# Autodesk Inventor assembly: teljes3
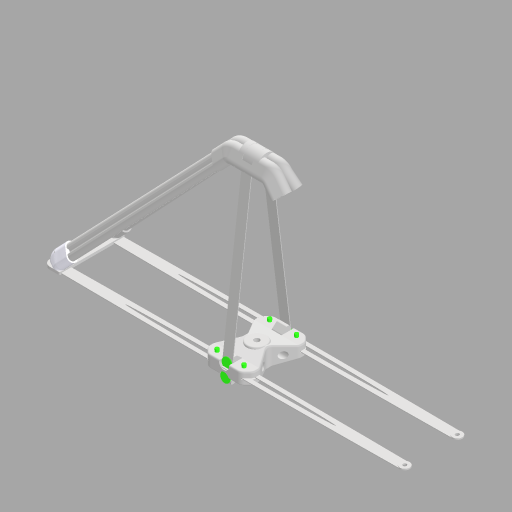
[picture p0: Inventor's stored thumbnail of the model, 512x512]
Saved by Autodesk Inventor 2023 (Build 270158000, 158)
## iProperties
Created: 2022-11-11
Part Number: teljes3
Document SubType Name: Assembly
Designer: gd1
Author: gd1
## Documents named in this file (8)
- C:\Users\gd1\3D Objects\3D nagyteherbírású híd\Híd\H-d\teljes8.iam
- C:\Users\gd1\3D Objects\3D nagyteherbírású híd\Híd\H-d\45 fok középre_talp másolata.ipt
- C:\Users\gd1\3D Objects\3D nagyteherbírású híd\Híd\H-d\palca 325mm.ipt
- C:\Users\gd1\3D Objects\3D nagyteherbírású híd\Híd\H-d\kozepcsati2.iam
- C:\Users\gd1\3D Objects\3D nagyteherbírású híd\Híd\H-d\szalag5.ipt
- C:\Users\gd1\3D Objects\3D nagyteherbírású híd\Híd\H-d\kozepso_csomopont2.0.ipt
- C:\Users\gd1\3D Objects\3D nagyteherbírású híd\Híd\H-d\szalag3.ipt
- C:\Users\gd1\3D Objects\3D nagyteherbírású híd\Híd\H-d\tipli.ipt
## Components (18 placed, 7 different names)
1. 45 fok középre_talp másolata:1 — Rotational:1, Rotational:2, Rigid:1, Rotational:4
2. palca 325mm:1 — Rotational:1
3. palca 325mm:2 — Rotational:2, Mate:1
4. kozepcsati2:1 [sub-assembly] — Mate:1, Mate:2
5. szalag5:1 — Mate:2, Rotational:3, Rigid:2, Rigid:3, Rigid:4, Rigid:5
6. kozepso_csomopont2.0:1 — Rotational:3
7. szalag3:1 — Rigid:1, Rotational:5, Rotational:6, Rotational:10
8. szalag3:2 — Rotational:4, Rotational:7, Rotational:8, Rotational:9
9. tipli:1 — Rigid:2
10. tipli:2 — Rigid:3
11. tipli:3 — Rigid:4
12. tipli:4 — Rigid:5
13. tipli:5 — Rotational:5
14. tipli:6 — Rotational:6
15. tipli:7 — Rotational:7
16. tipli:8 — Rotational:8
17. tipli:9 — Rotational:9
18. tipli:10 — Rotational:10
## Relationships (17: RevoluteJoint 10, WeldJoint 5, Mate 2)
- Rotational:1 [RevoluteJoint]: 45 fok középre_talp másolata:1 ↔ palca 325mm:1
- Rotational:2 [RevoluteJoint]: 45 fok középre_talp másolata:1 ↔ palca 325mm:2
- Mate:1: palca 325mm:2 ↔ kozepcsati2:1
- Mate:2: kozepcsati2:1 ↔ szalag5:1
- Rotational:3 [RevoluteJoint]: szalag5:1 ↔ kozepso_csomopont2.0:1
- Rigid:1 [WeldJoint]: 45 fok középre_talp másolata:1 ↔ szalag3:1
- Rotational:4 [RevoluteJoint]: 45 fok középre_talp másolata:1 ↔ szalag3:2
- Rigid:2 [WeldJoint]: szalag5:1 ↔ tipli:1
- Rigid:3 [WeldJoint]: szalag5:1 ↔ tipli:2
- Rigid:4 [WeldJoint]: szalag5:1 ↔ tipli:3
- Rigid:5 [WeldJoint]: szalag5:1 ↔ tipli:4
- Rotational:5 [RevoluteJoint]: szalag3:1 ↔ tipli:5
- Rotational:6 [RevoluteJoint]: szalag3:1 ↔ tipli:6
- Rotational:7 [RevoluteJoint]: szalag3:2 ↔ tipli:7
- Rotational:8 [RevoluteJoint]: szalag3:2 ↔ tipli:8
- Rotational:9 [RevoluteJoint]: szalag3:2 ↔ tipli:9
- Rotational:10 [RevoluteJoint]: szalag3:1 ↔ tipli:10
